# Autodesk Inventor assembly: y_carriage_assembly
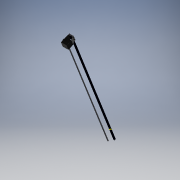
[picture p0: Inventor's stored thumbnail of the model, 180x180]
Saved by Autodesk Inventor 2018 (Build 220112000, 112)
## iProperties
Created: 2017-11-16
Part Number: y_carriage_assembly
Document SubType Name: Assembly
Designer: g
Author: g
## Documents named in this file (8)
- C:\Users\g\Desktop\AUG_inventor\y_carriage_assembly.iam
- C:\Users\g\Desktop\AUG_inventor\M3 X 10mm Screw.ipt
- C:\Users\g\Desktop\AUG_inventor\NEMA17 w connector metric.ipt
- C:\Users\g\Desktop\AUG_inventor\8M 900mm threaded rod.ipt
- C:\Users\g\Desktop\AUG_inventor\makerbeam1000mm.ipt
- C:\Users\g\Desktop\AUG_inventor\5mm to 8mm holder.ipt
- C:\Users\g\Desktop\AUG_inventor\makerbeam40mm.ipt
- C:\Users\g\Desktop\AUG_inventor\nema 17 holder.ipt
## Components (13 placed, 7 different names)
1. 8M 900mm threaded rod:1 — Rigid:8, Mate:290, Mate:291, Mate:292
2. makerbeam1000mm:1 — Flush:172, Mate:288, Mate:289, Flush:173, Flush:174, Flush:175, Flush:176
3. NEMA17 w connector metric:4 — Flush:172, Mate:290, Mate:291, Mate:292
4. 5mm to 8mm holder:1 — Rigid:8
5. makerbeam40mm:1 — Mate:288, Flush:174, Flush:175, Flush:177, Flush:178
6. makerbeam40mm:2 — Mate:289, Flush:173, Flush:176, Mate:293
7. nema 17 holder:1 — Flush:177, Flush:178, Mate:293, Cylindrical:124, Cylindrical:125, Cylindrical:126, Mate:294, Mate:295, Mate:296, Cylindrical:127, Cylindrical:128, Cylindrical:129, Mate:297, Mate:298, Mate:299
8. M3 X 10mm Screw:53 — Cylindrical:124, Mate:294
9. M3 X 10mm Screw:54 — Cylindrical:127, Mate:299
10. M3 X 10mm Screw:55 — Cylindrical:128, Mate:298
11. M3 X 10mm Screw:56 — Cylindrical:129, Mate:297
12. M3 X 10mm Screw:57 — Cylindrical:126, Mate:296
13. M3 X 10mm Screw:58 — Cylindrical:125, Mate:295
## Relationships (26: Mate 12, Flush 7, CylindricalJoint 6, WeldJoint 1)
- Rigid:8 [WeldJoint] (-12 mm): 8M 900mm threaded rod:1 ↔ 5mm to 8mm holder:1
- Flush:172: makerbeam1000mm:1 ↔ NEMA17 w connector metric:4
- Mate:288: makerbeam1000mm:1 ↔ makerbeam40mm:1
- Mate:289: makerbeam1000mm:1 ↔ makerbeam40mm:2
- Flush:173: makerbeam1000mm:1 ↔ makerbeam40mm:2
- Flush:174: makerbeam1000mm:1 ↔ makerbeam40mm:1
- Flush:175: makerbeam1000mm:1 ↔ makerbeam40mm:1
- Flush:176: makerbeam1000mm:1 ↔ makerbeam40mm:2
- Mate:290: 8M 900mm threaded rod:1 ↔ NEMA17 w connector metric:4
- Mate:291: 8M 900mm threaded rod:1 ↔ NEMA17 w connector metric:4
- Mate:292: 8M 900mm threaded rod:1 ↔ NEMA17 w connector metric:4
- Flush:177: makerbeam40mm:1 ↔ nema 17 holder:1
- Flush:178: makerbeam40mm:1 ↔ nema 17 holder:1
- Mate:293: makerbeam40mm:2 ↔ nema 17 holder:1
- Cylindrical:124: nema 17 holder:1 ↔ M3 X 10mm Screw:53
- Cylindrical:125: nema 17 holder:1 ↔ M3 X 10mm Screw:58
- Cylindrical:126: nema 17 holder:1 ↔ M3 X 10mm Screw:57
- Mate:294: nema 17 holder:1 ↔ M3 X 10mm Screw:53
- Mate:295: nema 17 holder:1 ↔ M3 X 10mm Screw:58
- Mate:296: nema 17 holder:1 ↔ M3 X 10mm Screw:57
- Cylindrical:127: nema 17 holder:1 ↔ M3 X 10mm Screw:54
- Cylindrical:128: nema 17 holder:1 ↔ M3 X 10mm Screw:55
- Cylindrical:129: nema 17 holder:1 ↔ M3 X 10mm Screw:56
- Mate:297: nema 17 holder:1 ↔ M3 X 10mm Screw:56
- Mate:298: nema 17 holder:1 ↔ M3 X 10mm Screw:55
- Mate:299: nema 17 holder:1 ↔ M3 X 10mm Screw:54
